# Autodesk Inventor assembly: Link2
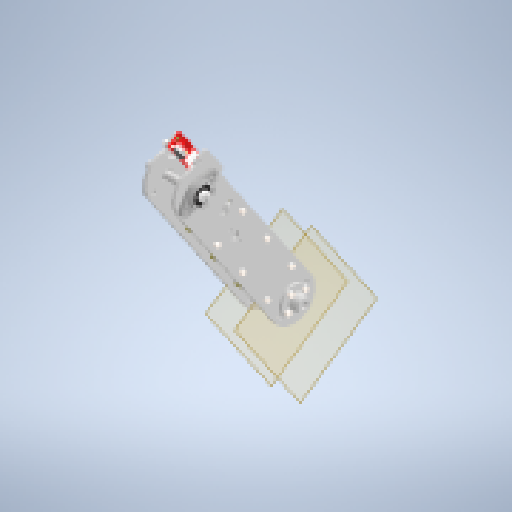
[picture p0: Inventor's stored thumbnail of the model, 512x512]
Saved by Autodesk Inventor 2023 (Build 270158000, 158)
## iProperties
Created: 2023-09-09
Part Number: Link2
Document SubType Name: Assembly
Designer: philo
Author: philo
## Documents named in this file (13)
- D:\02_3D_design_new\Link2.iam
- D:\02_3D_design_new\Link2Base.ipt
- D:\02_3D_design_new\goidoObi.ipt
- D:\02_3D_design_new\truc8mm.ipt
- D:\02_3D_design_new\GT2 Pulley 20 Tooth (ID6mm).ipt
- D:\02_3D_design_new\trudong3mm.ipt
- D:\02_3D_design_new\M3 x 5mm.ipt
- D:\02_3D_design_new\codinhtruc.ipt
- D:\02_3D_design_new\Dongco.iam
- D:\02_3D_design_new\limitswitch.ipt
- D:\02_3D_design_new\bulong5mmdai50.ipt
- D:\02_3D_design_new\oc5mm.ipt
- D:\02_3D_design_new\gt2smooth.ipt
## Components (43 placed, 12 different names)
1. M3 x 5mm:18 — Mate:146, Mate:147
2. M3 x 5mm:19 — Mate:148, Mate:149
3. M3 x 5mm:20 — Mate:152, Mate:155
4. M3 x 5mm:21 — Mate:150, Mate:156
5. M3 x 5mm:22 — Mate:151, Mate:154
6. M3 x 5mm:23 — Mate:153, Mate:157
7. M3 x 5mm:25 — Mate:161, Mate:162
8. M3 x 5mm:26 — Mate:160, Mate:165
9. M3 x 5mm:27 — Mate:159, Mate:164
10. M3 x 5mm:28 — Mate:158, Mate:163
11. limitswitch:2 — Mate:143, Flush:7, Mate:144, Mate:145
12. M3 x 5mm:17 — Mate:129, Mate:136
13. M3 x 5mm:16 — Mate:130, Mate:137
14. M3 x 5mm:15 — Mate:131, Mate:138
15. M3 x 5mm:14 — Mate:132, Mate:139
16. M3 x 5mm:13 — Mate:133, Mate:140
17. M3 x 5mm:12 — Mate:134, Mate:141
18. M3 x 5mm:7 — Mate:118, Mate:119
19. M3 x 5mm:6 — Mate:117, Mate:123
20. M3 x 5mm:5 — Mate:116, Mate:122
21. M3 x 5mm:4 — Mate:115, Mate:121
22. M3 x 5mm:2 — Mate:113, Mate:124
23. M3 x 5mm:1 — Mate:112, Mate:120
24. trudong3mm:9 — Mate:108, Mate:109, Mate:120
25. trudong3mm:8 — Mate:102, Mate:104
26. trudong3mm:7 — Mate:103, Mate:105, Mate:121
27. trudong3mm:3 — Mate:101, Mate:107
28. trudong3mm:2 — Mate:100, Mate:106, Mate:124
29. trudong3mm:1 — Mate:98, Mate:99
30. oc5mm:3 — Mate:96, Mate:97
31. oc5mm:2 — Mate:94, Mate:95
32. gt2smooth:1 — Mate:92, Mate:93
33. oc5mm:1 — Mate:90, Mate:91
34. GT2 Pulley 20 Tooth (ID6mm):1 — Mate:80, Mate:81
35. Dongco:1 [sub-assembly] — Mate:78, Angle:3, Mate:79, Mate:80
36. Link2Base:2 — Mate:71, Mate:72, Mate:73, Mate:74, Mate:75, Angle:2, Mate:78, Mate:79, Mate:81, Mate:88, Flush:6, Mate:89, Mate:90, Mate:93, Mate:98, Mate:99, Mate:100, Mate:101, Mate:102, Mate:103, Mate:104, Mate:105, Mate:106, Mate:107, Mate:108, Mate:109, Mate:129, Mate:130, Mate:131, Mate:132, Mate:133, Mate:134, Mate:136, Mate:137, Mate:138, Mate:139, Mate:140, Mate:141, Mate:143, Flush:7, Mate:144, Mate:145, Mate:146, Mate:147, Mate:148, Mate:149
37. Link2Base:3 — Mate:68, Mate:69, Mate:70, Angle:3, Mate:82, Mate:83, Mate:94, Mate:96, Mate:112, Mate:113, Mate:115, Mate:116, Mate:117, Mate:118, Mate:119, Mate:122, Mate:123, Mate:164
38. goidoObi:2
39. truc8mm:1
40. goidoObi:3 — Mate:74, Mate:75, Angle:2, Mate:82
41. codinhtruc:1 — Mate:68, Mate:69, Mate:70, Mate:158, Mate:159, Mate:160, Mate:161, Mate:162, Mate:163, Mate:165
42. codinhtruc:2 — Mate:71, Mate:72, Mate:73, Mate:83, Mate:150, Mate:151, Mate:152, Mate:153, Mate:154, Mate:155, Mate:156, Mate:157
43. bulong5mmdai50:1 — Mate:88, Flush:6, Mate:89, Mate:91, Mate:92, Mate:95, Mate:97
## Relationships (93: Mate 87, Angle 3, Flush 3)
- [Mate] (30 mm): Link2Base:2 ↔ Link2Base:3
- [Mate]: Link2Base:3 ↔ goidoObi:2
- [Mate]: Link2Base:3 ↔ goidoObi:2
- [Angle] (90 deg): Link2Base:3 ↔ goidoObi:2
- [Flush] (-5 mm): goidoObi:2 ↔ truc8mm:1
- [Mate]: goidoObi:2 ↔ truc8mm:1
- Mate:68: Link2Base:3 ↔ codinhtruc:1
- Mate:69: Link2Base:3 ↔ codinhtruc:1
- Mate:70: Link2Base:3 ↔ codinhtruc:1
- Mate:71: Link2Base:2 ↔ codinhtruc:2
- Mate:72: Link2Base:2 ↔ codinhtruc:2
- Mate:73: Link2Base:2 ↔ codinhtruc:2
- Mate:74: Link2Base:2 ↔ goidoObi:3
- Mate:75: Link2Base:2 ↔ goidoObi:3
- Angle:2 (0 deg): Link2Base:2 ↔ goidoObi:3
- Mate:78: Dongco:1 ↔ Link2Base:2
- Angle:3 (0 deg): Dongco:1 ↔ Link2Base:3
- Mate:79: Dongco:1 ↔ Link2Base:2
- Mate:80: GT2 Pulley 20 Tooth (ID6mm):1 ↔ Dongco:1
- Mate:81 (2 mm): GT2 Pulley 20 Tooth (ID6mm):1 ↔ Link2Base:2
- Mate:82: Link2Base:3 ↔ goidoObi:3
- Mate:83: Link2Base:3 ↔ codinhtruc:2
- Mate:88 (2.5 mm): Link2Base:2 ↔ bulong5mmdai50:1
- Flush:6 (15 mm): Link2Base:2 ↔ bulong5mmdai50:1
- Mate:89: Link2Base:2 ↔ bulong5mmdai50:1
- Mate:90: oc5mm:1 ↔ Link2Base:2
- Mate:91: oc5mm:1 ↔ bulong5mmdai50:1
- Mate:92: gt2smooth:1 ↔ bulong5mmdai50:1
- Mate:93 (8 mm): gt2smooth:1 ↔ Link2Base:2
- Mate:94: oc5mm:2 ↔ Link2Base:3
- Mate:95: oc5mm:2 ↔ bulong5mmdai50:1
- Mate:96: oc5mm:3 ↔ Link2Base:3
- Mate:97: oc5mm:3 ↔ bulong5mmdai50:1
- Mate:98: trudong3mm:1 ↔ Link2Base:2
- Mate:99: trudong3mm:1 ↔ Link2Base:2
- Mate:100: trudong3mm:2 ↔ Link2Base:2
- Mate:101: trudong3mm:3 ↔ Link2Base:2
- Mate:102: trudong3mm:8 ↔ Link2Base:2
- Mate:103: trudong3mm:7 ↔ Link2Base:2
- Mate:104: trudong3mm:8 ↔ Link2Base:2
- Mate:105: trudong3mm:7 ↔ Link2Base:2
- Mate:106: trudong3mm:2 ↔ Link2Base:2
- Mate:107: trudong3mm:3 ↔ Link2Base:2
- Mate:108: trudong3mm:9 ↔ Link2Base:2
- Mate:109: trudong3mm:9 ↔ Link2Base:2
- Mate:112: M3 x 5mm:1 ↔ Link2Base:3
- Mate:113: M3 x 5mm:2 ↔ Link2Base:3
- Mate:115: M3 x 5mm:4 ↔ Link2Base:3
- Mate:116: M3 x 5mm:5 ↔ Link2Base:3
- Mate:117: M3 x 5mm:6 ↔ Link2Base:3
- Mate:118: M3 x 5mm:7 ↔ Link2Base:3
- Mate:119: M3 x 5mm:7 ↔ Link2Base:3
- Mate:120: M3 x 5mm:1 ↔ trudong3mm:9
- Mate:121: M3 x 5mm:4 ↔ trudong3mm:7
- Mate:122: M3 x 5mm:5 ↔ Link2Base:3
- Mate:123: M3 x 5mm:6 ↔ Link2Base:3
- Mate:124: M3 x 5mm:2 ↔ trudong3mm:2
- Mate:129: M3 x 5mm:17 ↔ Link2Base:2
- Mate:130: M3 x 5mm:16 ↔ Link2Base:2
- Mate:131: M3 x 5mm:15 ↔ Link2Base:2
- Mate:132: M3 x 5mm:14 ↔ Link2Base:2
- Mate:133: M3 x 5mm:13 ↔ Link2Base:2
- Mate:134: M3 x 5mm:12 ↔ Link2Base:2
- Mate:136: M3 x 5mm:17 ↔ Link2Base:2
- Mate:137: M3 x 5mm:16 ↔ Link2Base:2
- Mate:138: M3 x 5mm:15 ↔ Link2Base:2
- Mate:139: M3 x 5mm:14 ↔ Link2Base:2
- Mate:140: M3 x 5mm:13 ↔ Link2Base:2
- Mate:141: M3 x 5mm:12 ↔ Link2Base:2
- Mate:143: limitswitch:2 ↔ Link2Base:2
- Flush:7: limitswitch:2 ↔ Link2Base:2
- Mate:144: limitswitch:2 ↔ Link2Base:2
- Mate:145: limitswitch:2 ↔ Link2Base:2
- Mate:146: M3 x 5mm:18 ↔ Link2Base:2
- Mate:147: M3 x 5mm:18 ↔ Link2Base:2
- Mate:148: M3 x 5mm:19 ↔ Link2Base:2
- Mate:149: M3 x 5mm:19 ↔ Link2Base:2
- Mate:150: M3 x 5mm:21 ↔ codinhtruc:2
- Mate:151: M3 x 5mm:22 ↔ codinhtruc:2
- Mate:152: M3 x 5mm:20 ↔ codinhtruc:2
- Mate:153: M3 x 5mm:23 ↔ codinhtruc:2
- Mate:154: M3 x 5mm:22 ↔ codinhtruc:2
- Mate:155: M3 x 5mm:20 ↔ codinhtruc:2
- Mate:156: M3 x 5mm:21 ↔ codinhtruc:2
- Mate:157: M3 x 5mm:23 ↔ codinhtruc:2
- Mate:158: M3 x 5mm:28 ↔ codinhtruc:1
- Mate:159: M3 x 5mm:27 ↔ codinhtruc:1
- Mate:160: M3 x 5mm:26 ↔ codinhtruc:1
- Mate:161: M3 x 5mm:25 ↔ codinhtruc:1
- Mate:162: M3 x 5mm:25 ↔ codinhtruc:1
- Mate:163: M3 x 5mm:28 ↔ codinhtruc:1
- Mate:164: M3 x 5mm:27 ↔ Link2Base:3
- Mate:165: M3 x 5mm:26 ↔ codinhtruc:1
